# Autodesk Inventor assembly: Сборка1
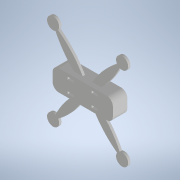
[picture p0: Inventor's stored thumbnail of the model, 180x180]
Saved by Autodesk Inventor 2022 (Build 260153000, 153)
## iProperties
Created: 2025-06-24
Part Number: Сборка1
Document SubType Name: Assembly
Designer: korsh524
Author: korsh524
## Documents named in this file (4)
- C:\git\Olymp20205Smena\Dezign\Drone\Сборка1.iam
- C:\git\Olymp20205Smena\Dezign\Drone\Dron.ipt
- C:\git\Olymp20205Smena\Dezign\Drone\bth.ipt
- C:\git\Olymp20205Smena\Dezign\Drone\top.ipt
## Components (6 placed, 3 different names)
1. Dron:1 — Заподлицо:1, Совмещение:2, Заподлицо:4, Заподлицо:5
2. bth:1 — Заподлицо:1, Совмещение:1, Заподлицо:2, Заподлицо:3
3. bth:2 — Совмещение:1, Заподлицо:2, Заподлицо:3
4. top:1 — Совмещение:2, Заподлицо:4, Заподлицо:5, Совмещение:3, Заподлицо:7, Заподлицо:9
5. top:2 — Совмещение:3, Совмещение:4, Заподлицо:6, Заподлицо:7, Заподлицо:8
6. top:3 — Совмещение:4, Заподлицо:6, Заподлицо:8, Заподлицо:9
## Relationships (13: Flush 9, Mate 4)
- Заподлицо:1 [Flush]: Dron:1 ↔ bth:1
- Совмещение:1 [Mate]: bth:1 ↔ bth:2
- Заподлицо:2 [Flush]: bth:1 ↔ bth:2
- Заподлицо:3 [Flush]: bth:1 ↔ bth:2
- Совмещение:2 [Mate]: Dron:1 ↔ top:1
- Заподлицо:4 [Flush]: Dron:1 ↔ top:1
- Заподлицо:5 [Flush]: Dron:1 ↔ top:1
- Совмещение:3 [Mate]: top:1 ↔ top:2
- Совмещение:4 [Mate]: top:2 ↔ top:3
- Заподлицо:6 [Flush]: top:2 ↔ top:3
- Заподлицо:7 [Flush]: top:1 ↔ top:2
- Заподлицо:8 [Flush]: top:2 ↔ top:3
- Заподлицо:9 [Flush]: top:1 ↔ top:3
